# Autodesk Inventor assembly: pneumatic_cylinder_assembly
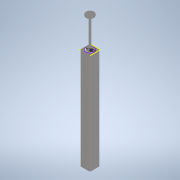
[picture p0: Inventor's stored thumbnail of the model, 180x180]
Saved by Autodesk Inventor 2022 (Build 260153000, 153)
## iProperties
Created: 2021-11-08
Part Number: pneumatic_cylinder_assembly
Document SubType Name: Assembly
Designer: kibandi
Author: kibandi
## Documents named in this file (3)
- C:\academics\YEAR 4\4.2\DOMS II\DOMS II projects\mechanical design\pneumatic_cylinder_assembly.iam
- C:\academics\YEAR 4\4.2\DOMS II\DOMS II projects\mechanical design\pneumatic_cylinder_ body.ipt
- C:\academics\YEAR 4\4.2\DOMS II\DOMS II projects\mechanical design\pneumatic_cylinder_rod.ipt
## Components (2 placed, 2 different names)
1. pneumatic_cylinder_ body:1 — Insert:1
2. pneumatic_cylinder_rod:1 — Insert:1
## Relationships (1: Insert 1)
- Insert:1: pneumatic_cylinder_ body:1 ↔ pneumatic_cylinder_rod:1
